# Autodesk Inventor assembly: TestingThingIVerseRPiZeroW
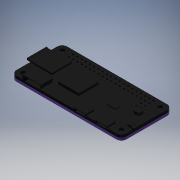
[picture p0: Inventor's stored thumbnail of the model, 180x180]
Saved by Autodesk Inventor 2019.2 (Build 232265000, 265)
## iProperties
Created: 2018-12-19
Part Number: TestingThingIVerseRPiZeroW
Document SubType Name: Assembly
Designer: steele
Author: steele
## Documents named in this file (3)
- C:\git\CAD-Development\robSteele\ShapeWays\TelescopeProjects\PiZeroWCamera\TestingThingIVerseRPiZeroW.iam
- C:\git\CAD-Development\robSteele\ShapeWays\TelescopeProjects\PiZeroWCamera\PiZeroWMechanicalLayout.ipt
- C:\git\CAD-Development\robSteele\ShapeWays\TelescopeProjects\PiZeroWCamera\Pi_Zero_W_ThingIVerse.ipt
## Components (2 placed, 2 different names)
1. PiZeroWMechanicalLayout:1 — Insert:1, Insert:2
2. Pi_Zero_W_ThingIVerse:1 — Insert:1, Insert:2
## Relationships (2: Insert 2)
- Insert:1: PiZeroWMechanicalLayout:1 ↔ Pi_Zero_W_ThingIVerse:1
- Insert:2: PiZeroWMechanicalLayout:1 ↔ Pi_Zero_W_ThingIVerse:1
